# Autodesk Inventor assembly: P25K1-Step
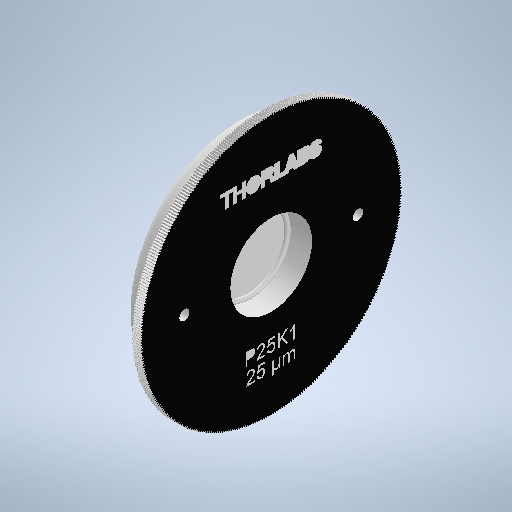
[picture p0: Inventor's stored thumbnail of the model, 512x512]
Saved by Autodesk Inventor 2025.2 (Build 292293000, 293)
## iProperties
Created: 2024-04-05
Part Number: P25K1-Step
Description: STEP AP203
Document SubType Name: Assembly
Designer: monolithic
Sending System: SolidWorks 2022
Preprocessor: SwSTEP 2.0
Title: TTN348089-E0W.STEP
Revision Number: ANY
## Documents named in this file (4)
- C:\Users\monolithic\Documents\GitHub\CAD\Monolith\John\Altair_PowellAndCylindricalBaseplatesCombined_10_16_2025\Assemblies\Subassemblies\P25K1-Step\P25K1-Step\P25K1-Step.iam
- C:\Users\monolithic\Documents\GitHub\CAD\Monolith\John\Altair_PowellAndCylindricalBaseplatesCombined_10_16_2025\Assemblies\Subassemblies\P25K1-Step\P25K1-Step\DWG2156.ipt
- C:\Users\monolithic\Documents\GitHub\CAD\Monolith\John\Altair_PowellAndCylindricalBaseplatesCombined_10_16_2025\Assemblies\Subassemblies\P25K1-Step\P25K1-Step\DWG2271_25µm.ipt
- C:\Users\monolithic\Documents\GitHub\CAD\Monolith\John\Altair_PowellAndCylindricalBaseplatesCombined_10_16_2025\Assemblies\Subassemblies\P25K1-Step\P25K1-Step\DWG2082_Design Only.ipt
## Components (3 placed, 3 different names)
1. DWG2156_1
2. DWG2271_25µm_2
3. DWG2082_Design Only_3
## Named parameters: Finish1_Area = 6.39115
note: some values were not read from the file. Shown as the stored number, unit unknown: "Finish1_Area".
